# Autodesk Inventor assembly: 01.02.03.00 - Braço esquerdo
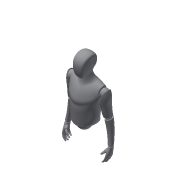
[picture p0: Inventor's stored thumbnail of the model, 180x180]
Saved by Autodesk Inventor 2016 (Build 200138000, 138)
## iProperties
Created: 2017-03-23
Part Number: 01.02.03.00 - Braço esquerdo
Document SubType Name: Assembly
Designer: Wesley Perez
Author: Wesley Perez
## Documents named in this file (5)
- D:\EMPRESARIAL\ADEBOTT\Dep. PROJETOS\ADEBOTT - KIT PROJETISTA\Corpos Humanos\Corpo Humano 01\Parts\01.02.01.00 - Membros superiores.iam
- D:\EMPRESARIAL\ADEBOTT\Dep. PROJETOS\ADEBOTT - KIT PROJETISTA\Corpos Humanos\Corpo Humano 01\Parts\01.02.01.01 - Torso.ipt
- D:\EMPRESARIAL\ADEBOTT\Dep. PROJETOS\ADEBOTT - KIT PROJETISTA\Corpos Humanos\Corpo Humano 01\Parts\01.02.01.02 - Cabeça.ipt
- D:\EMPRESARIAL\ADEBOTT\Dep. PROJETOS\ADEBOTT - KIT PROJETISTA\Corpos Humanos\Corpo Humano 01\Parts\01.02.02.00 - Braço direito.iam
- D:\EMPRESARIAL\ADEBOTT\Dep. PROJETOS\ADEBOTT - KIT PROJETISTA\Corpos Humanos\Corpo Humano 01\Parts\01.02.03.00 - Braço esquerdo.iam
## Components (4 placed, 4 different names)
1. 01.02.01.01 - Torso:1 — Alinhamento:1, Alinhamento:2, Alinhamento:3, Coincidência:1, Coincidência:2, Coincidência:3
2. 01.02.01.02 - Cabeça:1 — Coincidência:1
3. 01.02.02.00 - Braço direito:1 [sub-assembly] — Coincidência:3
4. 01.02.03.00 - Braço esquerdo:1 [sub-assembly] — Coincidência:2
## Relationships (6: Flush 3, Mate 3)
- Alinhamento:1 [Flush]: 01.02.01.01 - Torso:1
- Alinhamento:2 [Flush]: 01.02.01.01 - Torso:1
- Alinhamento:3 [Flush]: 01.02.01.01 - Torso:1
- Coincidência:1 [Mate]: 01.02.01.01 - Torso:1 ↔ 01.02.01.02 - Cabeça:1
- Coincidência:2 [Mate]: 01.02.01.01 - Torso:1 ↔ 01.02.03.00 - Braço esquerdo:1
- Coincidência:3 [Mate]: 01.02.01.01 - Torso:1 ↔ 01.02.02.00 - Braço direito:1
